# Autodesk Inventor assembly: Y-axis Belt Idler assy
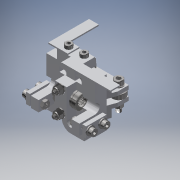
[picture p0: Inventor's stored thumbnail of the model, 180x180]
Saved by Autodesk Inventor 2018 (Build 220112000, 112)
## iProperties
Created: 2017-10-03
Part Number: Y-axis Belt Idler assy
Document SubType Name: Assembly
Designer: Gabriel Smolnycki
Author: Gabriel Smolnycki
## Documents named in this file (16)
- E:\planb\mechanics\Subassemblies\Y-axis Belt Idler assy.iam
- E:\planb\mechanics\Y-axis\Y-axis Frame Block.ipt
- E:\planb\mechanics\Hardware\M4 SS Nut.ipt
- E:\planb\mechanics\Hardware\8x25 Linear Bearing (63255K45).ipt
- E:\planb\mechanics\Hardware\4x13 SS Ball Bearing (7804K103).ipt
- E:\planb\mechanics\Hardware\M4x20 SS SHCS.ipt
- E:\planb\mechanics\Hardware\M4 SS Washer.ipt
- E:\planb\mechanics\Hardware\M4 SS Locknut.ipt
- E:\planb\mechanics\Y-axis\Y-axis Linear Bearing Clamp.ipt
- E:\planb\mechanics\Hardware\M4x35 SS SHCS.ipt
- E:\planb\mechanics\Y-axis\Y-axis Belt Clamp.ipt
- E:\planb\mechanics\Hardware\M4x16 SS SHCS.ipt
- E:\planb\mechanics\Y-axis\Y-axis Carriage Flag.ipt
- E:\planb\mechanics\Y-axis\Y-axis X-axis Flag.ipt
- E:\planb\mechanics\Y-axis\Y-axis Belt Idler.ipt
- E:\planb\mechanics\Hardware\M4x25 SS SHCS.ipt
## Components (49 placed, 15 different names)
1. Y-axis Frame Block:1 — Mate:1, Mate:2, Insert:1, Mate:3, Mate:4, Insert:2, Insert:3, Mate:5, Mate:6, Insert:4, Flush:1, Insert:5, Flush:2, Mate:7, Mate:8, Insert:20, Insert:21, Insert:22, Insert:35, Mate:9, Insert:36, Mate:10, Insert:37, Insert:38, Mate:11, Mate:12, Insert:43, Insert:44, Insert:45, Insert:46, Insert:47, Flush:3, Insert:49, Flush:4, Insert:51
2. M4 SS Nut:1 — Mate:1, Mate:2, Insert:1
3. M4 SS Nut:2 — Mate:3, Mate:4, Insert:2
4. 8x25 Linear Bearing (63255K45):1 — Insert:3
5. Y-axis Belt Idler:1 — Mate:5, Insert:4, Flush:1, Insert:6, Insert:8, Insert:10, Insert:11, Insert:12, Insert:13, Insert:27
6. Y-axis Belt Idler:2 — Mate:6, Insert:5, Flush:2, Insert:7, Insert:9, Insert:14, Insert:15, Insert:28
7. 4x13 SS Ball Bearing (7804K103):1 — Insert:8
8. 4x13 SS Ball Bearing (7804K103):2 — Insert:11
9. M4x25 SS SHCS:1
10. M4x25 SS SHCS:2
11. M4 SS Washer:1 — Insert:10
12. M4 SS Washer:2 — Insert:9
13. M4 SS Washer:3 — Insert:13
14. M4 SS Washer:4 — Insert:15, Insert:18
15. M4 SS Washer:5 — Insert:14, Insert:19
16. M4 SS Washer:6 — Insert:12
17. M4 SS Washer:7 — Insert:7
18. M4 SS Washer:8 — Insert:6
19. M4 SS Locknut:1 — Insert:18
20. M4 SS Locknut:2 — Insert:19
21. M4 SS Nut:3 — Mate:7, Mate:8, Insert:20
22. Y-axis Linear Bearing Clamp:1 — Insert:21, Insert:22, Insert:23, Insert:24
23. M4 SS Washer:9 — Insert:27
24. M4 SS Washer:10 — Insert:28
25. M4 SS Washer:11 — Insert:24, Insert:25
26. M4 SS Washer:12 — Insert:23, Insert:26
27. M4 SS Locknut:3 — Insert:25
28. M4 SS Locknut:4 — Insert:26
29. M4x35 SS SHCS:1
30. M4x35 SS SHCS:2
31. Y-axis Belt Clamp:1 — Insert:31, Insert:32, Insert:43, Insert:44
32. M4 SS Washer:13 — Insert:31, Insert:33
33. M4 SS Washer:14 — Insert:32, Insert:34
34. M4x20 SS SHCS:3 — Insert:33
35. M4x20 SS SHCS:4 — Insert:34
36. M4 SS Nut:4 — Insert:35, Mate:9
37. M4 SS Nut:5 — Insert:36, Mate:10
38. M4 SS Nut:6 — Insert:37, Mate:12
39. M4 SS Nut:7 — Insert:38, Mate:11
40. Y-axis Belt Clamp:2 — Insert:45, Insert:51
41. M4 SS Washer:15
42. M4 SS Washer:16
43. M4x20 SS SHCS:5
44. M4x20 SS SHCS:6
45. M4x16 SS SHCS:1 — Insert:46
46. M4x20 SS SHCS:7 — Insert:50
47. M4x20 SS SHCS:8 — Insert:48
48. Y-axis Carriage Flag:1 — Insert:47, Flush:3, Insert:48
49. Y-axis X-axis Flag:1 — Insert:49, Flush:4, Insert:50
## Relationships (67: Insert 51, Mate 12, Flush 4)
- Mate:1: Y-axis Frame Block:1 ↔ M4 SS Nut:1
- Mate:2: Y-axis Frame Block:1 ↔ M4 SS Nut:1
- Insert:1: Y-axis Frame Block:1 ↔ M4 SS Nut:1
- Mate:3: Y-axis Frame Block:1 ↔ M4 SS Nut:2
- Mate:4: Y-axis Frame Block:1 ↔ M4 SS Nut:2
- Insert:2: Y-axis Frame Block:1 ↔ M4 SS Nut:2
- Insert:3 (0.25 mm): Y-axis Frame Block:1 ↔ 8x25 Linear Bearing (63255K45):1
- Mate:5: Y-axis Frame Block:1 ↔ Y-axis Belt Idler:1
- Mate:6: Y-axis Frame Block:1 ↔ Y-axis Belt Idler:2
- Insert:4: Y-axis Frame Block:1 ↔ Y-axis Belt Idler:1
- Flush:1: Y-axis Frame Block:1 ↔ Y-axis Belt Idler:1
- Insert:5: Y-axis Frame Block:1 ↔ Y-axis Belt Idler:2
- Flush:2: Y-axis Frame Block:1 ↔ Y-axis Belt Idler:2
- Insert:6: Y-axis Belt Idler:1 ↔ M4 SS Washer:8
- Insert:7: Y-axis Belt Idler:2 ↔ M4 SS Washer:7
- Insert:8 (0.5 mm): Y-axis Belt Idler:1 ↔ 4x13 SS Ball Bearing (7804K103):1
- Insert:9: Y-axis Belt Idler:2 ↔ M4 SS Washer:2
- Insert:10: Y-axis Belt Idler:1 ↔ M4 SS Washer:1
- Insert:11 (0.5 mm): Y-axis Belt Idler:1 ↔ 4x13 SS Ball Bearing (7804K103):2
- Insert:12: Y-axis Belt Idler:1 ↔ M4 SS Washer:6
- Insert:13: Y-axis Belt Idler:1 ↔ M4 SS Washer:3
- Insert:14: Y-axis Belt Idler:2 ↔ M4 SS Washer:5
- Insert:15: Y-axis Belt Idler:2 ↔ M4 SS Washer:4
- [Insert]: M4x25 SS SHCS:1 ↔ M4 SS Washer:6
- [Insert]: M4x25 SS SHCS:2 ↔ M4 SS Washer:3
- Insert:18: M4 SS Washer:4 ↔ M4 SS Locknut:1
- Insert:19: M4 SS Washer:5 ↔ M4 SS Locknut:2
- Mate:7: Y-axis Frame Block:1 ↔ M4 SS Nut:3
- Mate:8: Y-axis Frame Block:1 ↔ M4 SS Nut:3
- Insert:20: Y-axis Frame Block:1 ↔ M4 SS Nut:3
- Insert:21: Y-axis Frame Block:1 ↔ Y-axis Linear Bearing Clamp:1
- Insert:22: Y-axis Frame Block:1 ↔ Y-axis Linear Bearing Clamp:1
- Insert:23: Y-axis Linear Bearing Clamp:1 ↔ M4 SS Washer:12
- Insert:24: Y-axis Linear Bearing Clamp:1 ↔ M4 SS Washer:11
- Insert:25: M4 SS Washer:11 ↔ M4 SS Locknut:3
- Insert:26: M4 SS Washer:12 ↔ M4 SS Locknut:4
- Insert:27: Y-axis Belt Idler:1 ↔ M4 SS Washer:9
- Insert:28: Y-axis Belt Idler:2 ↔ M4 SS Washer:10
- [Insert]: M4 SS Washer:9 ↔ M4x35 SS SHCS:1
- [Insert]: M4 SS Washer:10 ↔ M4x35 SS SHCS:2
- Insert:31: Y-axis Belt Clamp:1 ↔ M4 SS Washer:13
- Insert:32: Y-axis Belt Clamp:1 ↔ M4 SS Washer:14
- Insert:33: M4 SS Washer:13 ↔ M4x20 SS SHCS:3
- Insert:34: M4 SS Washer:14 ↔ M4x20 SS SHCS:4
- Insert:35: Y-axis Frame Block:1 ↔ M4 SS Nut:4
- Mate:9: Y-axis Frame Block:1 ↔ M4 SS Nut:4
- Insert:36: Y-axis Frame Block:1 ↔ M4 SS Nut:5
- Mate:10: Y-axis Frame Block:1 ↔ M4 SS Nut:5
- Insert:37: Y-axis Frame Block:1 ↔ M4 SS Nut:6
- Insert:38: Y-axis Frame Block:1 ↔ M4 SS Nut:7
- Mate:11: Y-axis Frame Block:1 ↔ M4 SS Nut:7
- Mate:12: Y-axis Frame Block:1 ↔ M4 SS Nut:6
- [Insert]: Y-axis Belt Clamp:2 ↔ M4 SS Washer:15
- [Insert]: Y-axis Belt Clamp:2 ↔ M4 SS Washer:16
- [Insert]: M4 SS Washer:15 ↔ M4x20 SS SHCS:5
- [Insert]: M4 SS Washer:16 ↔ M4x20 SS SHCS:6
- Insert:43 (2 mm): Y-axis Frame Block:1 ↔ Y-axis Belt Clamp:1
- Insert:44: Y-axis Frame Block:1 ↔ Y-axis Belt Clamp:1
- Insert:45 (2 mm): Y-axis Frame Block:1 ↔ Y-axis Belt Clamp:2
- Insert:46: Y-axis Frame Block:1 ↔ M4x16 SS SHCS:1
- Insert:47: Y-axis Frame Block:1 ↔ Y-axis Carriage Flag:1
- Flush:3: Y-axis Frame Block:1 ↔ Y-axis Carriage Flag:1
- Insert:48: M4x20 SS SHCS:8 ↔ Y-axis Carriage Flag:1
- Insert:49: Y-axis Frame Block:1 ↔ Y-axis X-axis Flag:1
- Flush:4: Y-axis Frame Block:1 ↔ Y-axis X-axis Flag:1
- Insert:50: M4x20 SS SHCS:7 ↔ Y-axis X-axis Flag:1
- Insert:51: Y-axis Frame Block:1 ↔ Y-axis Belt Clamp:2
## Named parameters: d62_d46 = 0 mm, d63_d47 = 0 mm, d64_d48 = 0 mm, d65_d49 = 0 mm
